# Autodesk Inventor assembly: OG prig assm
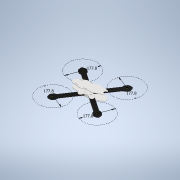
[picture p0: Inventor's stored thumbnail of the model, 180x180]
Saved by Autodesk Inventor 2020 (Build 240168000, 168)
## iProperties
Created: 2022-05-23
Part Number: OG prig assm
Document SubType Name: Assembly
Designer: Steven
Author: Steven
## Documents named in this file (4)
- Y:\FPV drone stuff\0 Street League\Frames\experimental-quad-frames\OG prig assm.iam
- Y:\FPV drone stuff\0 Street League\Frames\experimental-quad-frames\Kauri arm.ipt
- Y:\FPV drone stuff\0 Street League\Frames\experimental-quad-frames\399 prig z plate.ipt
- Y:\FPV drone stuff\0 Street League\Frames\experimental-quad-frames\399 prig top plate.ipt
## Components (7 placed, 3 different names)
1. Kauri arm:1 — Flush:3, Mate:1, Mate:2, Mate:6, Mate:11
2. Kauri arm:2 — Flush:2, Mate:3, Mate:9, Mate:12
3. Kauri arm:3 — Flush:1, Mate:4, Mate:8, Mate:10
4. Kauri arm:4 — Flush:1, Flush:2, Flush:3, Mate:5, Mate:7
5. 399 prig z plate:1 — Mate:1, Mate:2, Mate:3, Mate:4, Mate:5, Mate:6, Mate:7, Mate:8, Mate:9, Mate:14, Mate:15
6. 399 prig z plate:2 — Mate:10, Mate:11, Mate:12, Mate:13
7. 399 prig top plate:1 — Mate:13, Mate:14, Mate:15
## Relationships (18: Mate 15, Flush 3)
- Flush:1: Kauri arm:3 ↔ Kauri arm:4
- Flush:2: Kauri arm:2 ↔ Kauri arm:4
- Flush:3: Kauri arm:1 ↔ Kauri arm:4
- Mate:1: Kauri arm:1 ↔ 399 prig z plate:1
- Mate:2: Kauri arm:1 ↔ 399 prig z plate:1
- Mate:3: Kauri arm:2 ↔ 399 prig z plate:1
- Mate:4: Kauri arm:3 ↔ 399 prig z plate:1
- Mate:5: Kauri arm:4 ↔ 399 prig z plate:1
- Mate:6: Kauri arm:1 ↔ 399 prig z plate:1
- Mate:7: Kauri arm:4 ↔ 399 prig z plate:1
- Mate:8: Kauri arm:3 ↔ 399 prig z plate:1
- Mate:9: Kauri arm:2 ↔ 399 prig z plate:1
- Mate:10: Kauri arm:3 ↔ 399 prig z plate:2
- Mate:11: Kauri arm:1 ↔ 399 prig z plate:2
- Mate:12: Kauri arm:2 ↔ 399 prig z plate:2
- Mate:13 (25 mm): 399 prig z plate:2 ↔ 399 prig top plate:1
- Mate:14: 399 prig z plate:1 ↔ 399 prig top plate:1
- Mate:15: 399 prig z plate:1 ↔ 399 prig top plate:1
